# Autodesk Inventor assembly: Goal Rush
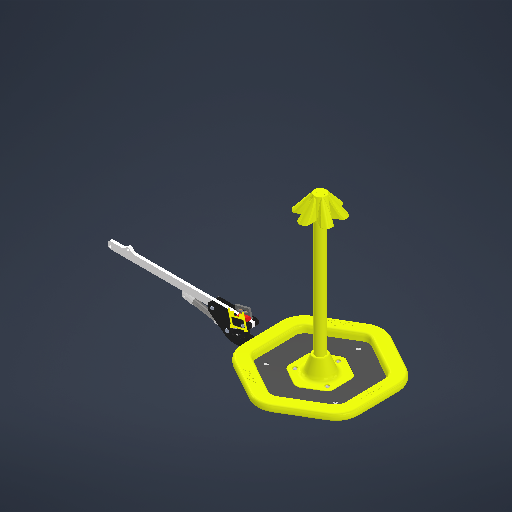
[picture p0: Inventor's stored thumbnail of the model, 512x512]
Saved by Autodesk Inventor 2025 (Build 290162000, 162)
## iProperties
Created: 2025-02-08
Part Number: Goal Rush
Document SubType Name: Assembly
Designer: Juan
Author: Juan
## Documents named in this file (19)
- C:\Users\Juan\Documents\GitHub\ATUM-VRC-High-Stakes-CAD\Protobot\Goal Rush.iam
- C:\Users\Juan\Documents\GitHub\ATUM-VRC-High-Stakes-CAD\Additional Parts\PolyCarb.ipt
- C:\Users\Juan\Documents\GitHub\ATUM-VRC-High-Stakes-CAD\Protobot\Goal Rush U Joint.ipt
- C:\Users\Juan\Documents\GitHub\ATUM-VRC-High-Stakes-CAD\VEX-CAD-Inventor\Motion\Pneumatics\Reference Parts\Pistons\25mm Stroke Pneumatic Cylinder Body.ipt
- C:\Users\Juan\Documents\GitHub\ATUM-VRC-High-Stakes-CAD\VEX-CAD-Inventor\Motion\Pneumatics\Reference Parts\Pistons\25mm Stroke Pneumatic Cylinder Rod.ipt
- C:\Users\Juan\Documents\GitHub\ATUM-VRC-High-Stakes-CAD\VEX-CAD-Inventor\Structure\Standoff\Standoff .50.ipt
- C:\Users\Juan\Documents\GitHub\ATUM-VRC-High-Stakes-CAD\VEX-CAD-Inventor\Structure\Standoff.ipt
- C:\Users\Juan\Documents\GitHub\ATUM-VRC-High-Stakes-CAD\VEX-CAD-Inventor\Motion\Spacers\Washer Teflon\TWasher .375 OD x .06250.ipt
- C:\Users\Juan\Documents\GitHub\ATUM-VRC-High-Stakes-CAD\VEX-CAD-Inventor\Motion\Spacers\Washer Teflon.ipt
- C:\Users\Juan\Documents\GitHub\ATUM-VRC-High-Stakes-CAD\Protobot\Goal Jaw Chassis Outer.ipt
- C:\Users\Juan\Documents\GitHub\ATUM-VRC-High-Stakes-CAD\Protobot\Goal Jaw Chassis Inner.ipt
- C:\Users\Juan\Documents\GitHub\ATUM-VRC-High-Stakes-CAD\VEX-CAD-Inventor\Structure\Hardware\Screw Steel - Star\SScrew Star Smooth .875.ipt
- C:\Users\Juan\Documents\GitHub\ATUM-VRC-High-Stakes-CAD\VEX-CAD-Inventor\Structure\Hardware\Screw Steel - Star.ipt
- C:\Users\Juan\Documents\GitHub\ATUM-VRC-High-Stakes-CAD\VEX-CAD-Inventor\Structure\Hardware\Nut Thin Nylock.ipt
- C:\Users\Juan\Documents\GitHub\ATUM-VRC-High-Stakes-CAD\VEX-CAD-Inventor\Structure\Hardware\Coupler\Coupler Star .5.ipt
- C:\Users\Juan\Documents\GitHub\ATUM-VRC-High-Stakes-CAD\VEX-CAD-Inventor\Structure\Hardware\Coupler.ipt
- C:\Users\Juan\Documents\GitHub\ATUM-VRC-High-Stakes-CAD\VEX-CAD-Inventor\Electronics\Sensors\Limit Switch.ipt
- C:\Users\Juan\Documents\GitHub\ATUM-VRC-High-Stakes-CAD\Protobot\Goal Jaw Tooth v4.ipt
- C:\Users\Juan\Documents\GitHub\ATUM-VRC-High-Stakes-CAD\Mobile Goal\276-8868-200.iam
## Components (20 placed, 14 different names)
1. PolyCarb:1 — Mate:6, Flush:3, Mate:16, Mate:17, Mate:18, Mate:19, Mate:20, Mate:21
2. Goal Jaw Tooth v4:1 — Mate:9, Mate:22, Mate:23
3. Goal Rush U Joint:1 — Mate:8, Flush:4, Mate:9, Mate:24
4. 25mm Stroke Pneumatic Cylinder Body:1 — Mate:6, Flush:3, Mate:7
5. 25mm Stroke Pneumatic Cylinder Rod:1 — Mate:7, Mate:8, Flush:4
6. Standoff .50:1 — Mate:12, Mate:13, Mate:14
7. TWasher .375 OD x .06250:1 — Mate:13, Mate:14
8. TWasher .375 OD x .06250:2 — Mate:12
9. Goal Jaw Chassis Outer:1 — Mate:16, Mate:17, Mate:18, Mate:23, Rigid:1, Rigid:2, Rigid:3, Rigid:4
10. Goal Jaw Chassis Inner:1 — Mate:19, Mate:20, Mate:21, Mate:22, Rigid:5, Rotational:1, Rigid:6
11. SScrew Star Smooth .875:1 — Rigid:2
12. SScrew Star Smooth .875:2 — Rigid:3
13. SScrew Star Smooth .875:3 — Rigid:1
14. SScrew Star Smooth .875:4 — Rigid:4
15. Nut Thin Nylock:1 — Rigid:5
16. Nut Thin Nylock:2 — Rotational:1
17. Nut Thin Nylock:3 — Rigid:6
18. Coupler Star .5:1 — Mate:24
19. Limit Switch:1
20. 276-8868-200:1 [sub-assembly]
## Relationships (25: Mate 16, WeldJoint 6, Flush 2, RevoluteJoint 1)
- Mate:6: PolyCarb:1 ↔ 25mm Stroke Pneumatic Cylinder Body:1
- Flush:3 (-2.8194 mm): PolyCarb:1 ↔ 25mm Stroke Pneumatic Cylinder Body:1
- Mate:7: 25mm Stroke Pneumatic Cylinder Body:1 ↔ 25mm Stroke Pneumatic Cylinder Rod:1
- Mate:8: Goal Rush U Joint:1 ↔ 25mm Stroke Pneumatic Cylinder Rod:1
- Flush:4: Goal Rush U Joint:1 ↔ 25mm Stroke Pneumatic Cylinder Rod:1
- Mate:9: Goal Jaw Tooth v4:1 ↔ Goal Rush U Joint:1
- Mate:12: Standoff .50:1 ↔ TWasher .375 OD x .06250:2
- Mate:13: Standoff .50:1 ↔ TWasher .375 OD x .06250:1
- Mate:14: Standoff .50:1 ↔ TWasher .375 OD x .06250:1
- Mate:16: PolyCarb:1 ↔ Goal Jaw Chassis Outer:1
- Mate:17: PolyCarb:1 ↔ Goal Jaw Chassis Outer:1
- Mate:18: PolyCarb:1 ↔ Goal Jaw Chassis Outer:1
- Mate:19: PolyCarb:1 ↔ Goal Jaw Chassis Inner:1
- Mate:20: PolyCarb:1 ↔ Goal Jaw Chassis Inner:1
- Mate:21: PolyCarb:1 ↔ Goal Jaw Chassis Inner:1
- Mate:22: Goal Jaw Tooth v4:1 ↔ Goal Jaw Chassis Inner:1
- Mate:23 (0.3969 mm): Goal Jaw Tooth v4:1 ↔ Goal Jaw Chassis Outer:1
- Rigid:1 [WeldJoint]: Goal Jaw Chassis Outer:1 ↔ SScrew Star Smooth .875:3
- Rigid:2 [WeldJoint]: Goal Jaw Chassis Outer:1 ↔ SScrew Star Smooth .875:1
- Rigid:3 [WeldJoint]: Goal Jaw Chassis Outer:1 ↔ SScrew Star Smooth .875:2
- Rigid:4 [WeldJoint]: Goal Jaw Chassis Outer:1 ↔ SScrew Star Smooth .875:4
- Rigid:5 [WeldJoint]: Goal Jaw Chassis Inner:1 ↔ Nut Thin Nylock:1
- Rotational:1 [RevoluteJoint]: Goal Jaw Chassis Inner:1 ↔ Nut Thin Nylock:2
- Rigid:6 [WeldJoint]: Goal Jaw Chassis Inner:1 ↔ Nut Thin Nylock:3
- Mate:24: Goal Rush U Joint:1 ↔ Coupler Star .5:1
